# Autodesk Inventor assembly: fischer price 20-1 reduction_mw
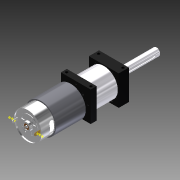
[picture p0: Inventor's stored thumbnail of the model, 180x180]
Saved by Autodesk Inventor 2011 (Build 150239000, 239)
## iProperties
Created: 2010-02-09
Part Number: fischer price 20-1 reduction_mw
Document SubType Name: Assembly
Designer: a
Author: a
## Documents named in this file (5)
- R:\2012\Inventor\vkop\All_Motors\fischer price 20-1 reduction_mw.iam
- R:\2012\Inventor\vkop\All_Motors\banebot 20-1 fischer price.ipt
- R:\2012\Inventor\vkop\All_Motors\Motors_BaneBots_RS-550.ipt
- \\lmss\STUDENTS\Robotics\Inventor\I_Team\Frame\Frame_Parts\mini winch motor bracket.ipt
- \\lmss\STUDENTS\Robotics\Inventor\I_Team\telescoping pole\mini winch pulley.ipt
## Components (4 placed, 4 different names)
1. banebot 20-1 fischer price:1 — Mate:1, Mate:2, Mate:3, Mate:4, Mate:5, Insert:1
2. Motors_BaneBots_RS-550:1 — Mate:1, Mate:2
3. mini winch motor bracket:1 — Mate:3, Mate:4, Mate:5
4. mini winch pulley:1 — Insert:1
## Relationships (6: Mate 5, Insert 1)
- Mate:1: banebot 20-1 fischer price:1 ↔ Motors_BaneBots_RS-550:1
- Mate:2: banebot 20-1 fischer price:1 ↔ Motors_BaneBots_RS-550:1
- Mate:3: banebot 20-1 fischer price:1 ↔ mini winch motor bracket:1
- Mate:4: banebot 20-1 fischer price:1 ↔ mini winch motor bracket:1
- Mate:5: banebot 20-1 fischer price:1 ↔ mini winch motor bracket:1
- Insert:1: banebot 20-1 fischer price:1 ↔ mini winch pulley:1
